# Autodesk Inventor assembly: phone-stand-assembly
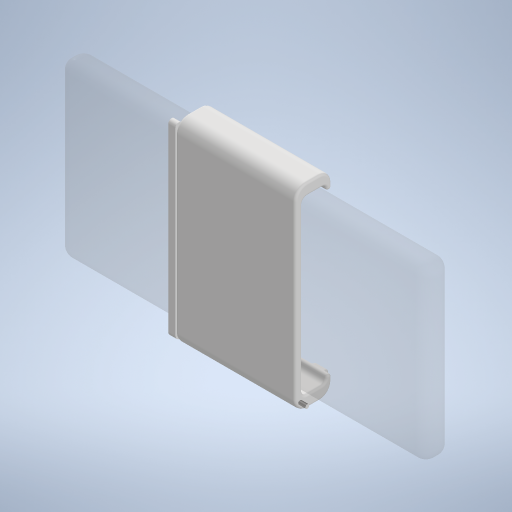
[picture p0: Inventor's stored thumbnail of the model, 512x512]
Saved by Autodesk Inventor 2023 (Build 270158030, 158C)
## iProperties
Created: 2023-04-28
Part Number: phone-stand-assembly
Document SubType Name: Assembly
Designer: Imogen Heard
Author: Imogen Heard
## Documents named in this file (5)
- C:\Users\dheard\Documents\0004-inventor\3D_CAD_Master\phone-holder\phone-stand-assembly.iam
- C:\Users\dheard\Documents\0004-inventor\3D_CAD_Master\phone-holder\samsung-s20.ipt
- C:\Users\dheard\Documents\0004-inventor\3D_CAD_Master\phone-holder\s20-phone-clip.ipt
- C:\Users\dheard\Documents\0004-inventor\3D_CAD_Master\phone-holder\pin.ipt
- C:\Users\dheard\Documents\0000.KiCad\Projects\000-personal-projects\esp32-faerfly\3D-cad\esp32-faerfly-inventor\case-stls\flip-stand-bottom.ipt
## Components (4 placed, 4 different names)
1. samsung-s20:1 — Flush:1, Flush:2
2. s20-phone-clip:1 — Flush:1, Flush:2, Flush:3, Flush:4, Flush:5, Flush:6
3. pin:1 — Flush:3, Flush:4
4. flip-stand-bottom:1 — Flush:5, Flush:6
## Relationships (6: Flush 6)
- Flush:1: samsung-s20:1 ↔ s20-phone-clip:1
- Flush:2: samsung-s20:1 ↔ s20-phone-clip:1
- Flush:3: s20-phone-clip:1 ↔ pin:1
- Flush:4: s20-phone-clip:1 ↔ pin:1
- Flush:5: s20-phone-clip:1 ↔ flip-stand-bottom:1
- Flush:6: s20-phone-clip:1 ↔ flip-stand-bottom:1
